# Autodesk Inventor assembly: Linear Actuator
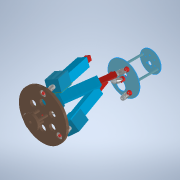
[picture p0: Inventor's stored thumbnail of the model, 180x180]
Saved by Autodesk Inventor 2021 (Build 250183000, 183)
## iProperties
Created: 2021-08-22
Part Number: Linear Actuator
Document SubType Name: Assembly
Designer: techv
Mass: 1736.04 g
Surface Area: 2681.18 cm^2
Volume: 406.885 cm^3
Density: 4.26665 g/cm^3
Author: techv
## Documents named in this file (17)
- D:\Projects\P_Borewell\V3\Linear Actuator.iam
- D:\Projects\P_Borewell\V3\Cylinder.ipt
- D:\Projects\P_Borewell\V3\plunger.ipt
- D:\Projects\P_Borewell\V3\lead screw.ipt
- D:\Projects\P_Borewell\V3\BRACKET N-20 motor v2_Predeterminado.ipt
- D:\Projects\P_Borewell\V3\MicroGearmotor v3.ipt.ipt
- D:\Projects\P_Borewell\V3\as 1420 - 1973 - m3 x 6.ipt
- D:\Projects\P_Borewell\V3\Part5^Assem1 N20 motor and flange.ipt
- D:\Projects\P_Borewell\V2\Design\sps manipulator\coupler.ipt
- D:\Projects\P_Borewell\V2\Design\sps manipulator\Bearing3.iam
- C:\Users\techv\Documents\Inventor\Content Center Files\R2021\en-US\AS 1474(1)\AS 1474 - M6(1).ipt
- C:\Users\techv\Documents\Capsule.ipt
- D:\Projects\P_Borewell\V2\Design\sps manipulator\Craftsman Socket U-Joint_2.iam
- D:\Projects\P_Borewell\V2\Design\sps manipulator\female joint for uv.ipt
- D:\Projects\P_Borewell\V2\Design\sps manipulator\base.ipt
- D:\Projects\P_Borewell\V2\Design\sps manipulator\platform.ipt
- MicroGearmotor v3.ipt
## Components (57 placed, 15 different names)
1. Cylinder:1 — Flush:1, Angle:1, Mate:19, Mate:25, Mate:35, Flush:6, Mate:36, Flush:7, Mate:61, Mate:62
2. plunger:1 — Mate:25, Flush:5, Mate:33, Mate:34, Mate:36, Mate:132, Mate:133
3. lead screw:1 — Flush:1, Mate:16, Mate:31, Mate:33
4. BRACKET N-20 motor v2_Predeterminado:1 — Flush:2, Mate:5, Mate:6, Mate:8, Mate:11, Mate:14, Mate:15
5. MicroGearmotor v3.ipt:1 — Mate:11, Mate:12, Mate:13, Mate:16, Mate:17, Mate:18
6. as 1420 - 1973 - m3 x 6:1 — Mate:5, Mate:6, Mate:7
7. as 1420 - 1973 - m3 x 6:2 — Mate:10, Mate:14, Mate:15
8. Part5^Assem1 N20 motor and flange:1 — Flush:2, Mate:7, Mate:8, Mate:10, Mate:12, Mate:13, Angle:1
9. coupler:1 — Mate:17, Mate:18, Mate:19, Mate:20
10. Bearing3:1 [sub-assembly] — Mate:20, Mate:35, Flush:6
11. AS 1474 - Metric M6:1 — Mate:31, Flush:5, Mate:34
12. Capsule:1 — Flush:7, Mate:60, Mate:61, Mate:62, Mate:109
13. Craftsman Socket U-Joint_2:2 [sub-assembly] — Mate:44, Mate:45, Mate:54, Mate:58
14. female joint for uv:4 — Mate:44, Mate:45, Mate:111, Mate:113
15. base:1 — Mate:37, Mate:38, Mate:39, Flush:8, Flush:9, Flush:10, Mate:55, Mate:57, Mate:58, Mate:59
16. Bearing3:2 [sub-assembly] — Mate:39, Flush:8, Mate:54
17. Bearing3:3 [sub-assembly] — Mate:38, Flush:10, Mate:53
18. Bearing3:4 [sub-assembly] — Mate:37, Flush:9, Mate:52, Mate:56
19. Craftsman Socket U-Joint_2:8 [sub-assembly] — Mate:55, Mate:57
20. female joint for uv:5
21. Craftsman Socket U-Joint_2:9 [sub-assembly] — Mate:52, Mate:56
22. female joint for uv:6 — Mate:60, Mate:109
23. Craftsman Socket U-Joint_2:10 [sub-assembly] — Mate:53, Mate:59
24. female joint for uv:7 — Mate:110, Mate:112
25. Cylinder:2
26. plunger:2 — Mate:130, Mate:131
27. lead screw:2
28. BRACKET N-20 motor v2_Predeterminado:2
29. MicroGearmotor v3.ipt:2
30. as 1420 - 1973 - m3 x 6:3
31. as 1420 - 1973 - m3 x 6:4
32. Part5^Assem1 N20 motor and flange:2
33. coupler:2
34. Bearing3:5 [sub-assembly]
35. AS 1474 - Metric M6:2
36. Capsule:2 — Mate:110, Mate:112
37. Cylinder:3
38. plunger:3 — Mate:134
39. lead screw:3
40. BRACKET N-20 motor v2_Predeterminado:3
41. MicroGearmotor v3.ipt:3
42. as 1420 - 1973 - m3 x 6:5
43. as 1420 - 1973 - m3 x 6:6
44. Part5^Assem1 N20 motor and flange:3
45. coupler:3
46. Bearing3:6 [sub-assembly]
47. AS 1474 - Metric M6:3
48. Capsule:3 — Mate:111, Mate:113
49. platform:1 — Mate:120, Mate:121, Mate:122, Mate:123, Mate:124, Mate:125, Mate:128, Mate:129
50. Craftsman Socket U-Joint_2:11 [sub-assembly] — Mate:122, Mate:123
51. female joint for uv:8 — Mate:132, Mate:133
52. Craftsman Socket U-Joint_2:12 [sub-assembly] — Mate:121, Mate:125
53. female joint for uv:9 — Mate:134
54. Craftsman Socket U-Joint_2:13 [sub-assembly] — Mate:120, Mate:124
55. female joint for uv:10 — Mate:130, Mate:131
56. Craftsman Socket U-Joint_2:14 [sub-assembly] — Mate:128, Mate:129
57. female joint for uv:11
## Relationships (136: Mate 115, Flush 18, Angle 3)
- Flush:1 (-5 mm): Cylinder:1 ↔ lead screw:1
- Flush:2: BRACKET N-20 motor v2_Predeterminado:1 ↔ Part5^Assem1 N20 motor and flange:1
- Mate:5: BRACKET N-20 motor v2_Predeterminado:1 ↔ as 1420 - 1973 - m3 x 6:1
- Mate:6: BRACKET N-20 motor v2_Predeterminado:1 ↔ as 1420 - 1973 - m3 x 6:1
- Mate:7: as 1420 - 1973 - m3 x 6:1 ↔ Part5^Assem1 N20 motor and flange:1
- Mate:8: BRACKET N-20 motor v2_Predeterminado:1 ↔ Part5^Assem1 N20 motor and flange:1
- Mate:10: as 1420 - 1973 - m3 x 6:2 ↔ Part5^Assem1 N20 motor and flange:1
- Mate:11: BRACKET N-20 motor v2_Predeterminado:1 ↔ MicroGearmotor v3.ipt:1
- Mate:12: MicroGearmotor v3.ipt:1 ↔ Part5^Assem1 N20 motor and flange:1
- Mate:13: MicroGearmotor v3.ipt:1 ↔ Part5^Assem1 N20 motor and flange:1
- Mate:14: BRACKET N-20 motor v2_Predeterminado:1 ↔ as 1420 - 1973 - m3 x 6:2
- Mate:15: BRACKET N-20 motor v2_Predeterminado:1 ↔ as 1420 - 1973 - m3 x 6:2
- Mate:16: lead screw:1 ↔ MicroGearmotor v3.ipt:1
- Angle:1 (0 deg): Cylinder:1 ↔ Part5^Assem1 N20 motor and flange:1
- Mate:17 (3 mm): MicroGearmotor v3.ipt:1 ↔ coupler:1
- Mate:18: MicroGearmotor v3.ipt:1 ↔ coupler:1
- Mate:19 (-5 mm): Cylinder:1 ↔ coupler:1
- Mate:20: coupler:1 ↔ Bearing3:1
- Mate:25: Cylinder:1 ↔ plunger:1
- Mate:31: lead screw:1 ↔ AS 1474 - Metric M6:1
- Flush:5: plunger:1 ↔ AS 1474 - Metric M6:1
- Mate:33: plunger:1 ↔ lead screw:1
- Mate:34: plunger:1 ↔ AS 1474 - Metric M6:1
- Mate:35: Cylinder:1 ↔ Bearing3:1
- Flush:6: Cylinder:1 ↔ Bearing3:1
- Mate:36: Cylinder:1 ↔ plunger:1
- Flush:7: Cylinder:1 ↔ Capsule:1
- Mate:37: base:1 ↔ Bearing3:4
- Mate:38: base:1 ↔ Bearing3:3
- Mate:39: base:1 ↔ Bearing3:2
- Flush:8: base:1 ↔ Bearing3:2
- Flush:9: base:1 ↔ Bearing3:4
- Flush:10: base:1 ↔ Bearing3:3
- Mate:44: Craftsman Socket U-Joint_2:2 ↔ female joint for uv:4
- Mate:45: Craftsman Socket U-Joint_2:2 ↔ female joint for uv:4
- [Mate]: Craftsman Socket U-Joint_2:8 ↔ female joint for uv:5
- [Mate]: Craftsman Socket U-Joint_2:8 ↔ female joint for uv:5
- [Mate]: Craftsman Socket U-Joint_2:9 ↔ female joint for uv:6
- [Mate]: Craftsman Socket U-Joint_2:9 ↔ female joint for uv:6
- [Mate]: Craftsman Socket U-Joint_2:10 ↔ female joint for uv:7
- [Mate]: Craftsman Socket U-Joint_2:10 ↔ female joint for uv:7
- Mate:52: Bearing3:4 ↔ Craftsman Socket U-Joint_2:9
- Mate:53: Bearing3:3 ↔ Craftsman Socket U-Joint_2:10
- Mate:54: Craftsman Socket U-Joint_2:2 ↔ Bearing3:2
- Mate:55: base:1 ↔ Craftsman Socket U-Joint_2:8
- Mate:56: Bearing3:4 ↔ Craftsman Socket U-Joint_2:9
- Mate:57: base:1 ↔ Craftsman Socket U-Joint_2:8
- Mate:58: Craftsman Socket U-Joint_2:2 ↔ base:1
- Mate:59: base:1 ↔ Craftsman Socket U-Joint_2:10
- Mate:60: Capsule:1 ↔ female joint for uv:6
- Mate:61: Cylinder:1 ↔ Capsule:1
- Mate:62: Cylinder:1 ↔ Capsule:1
- [Flush] (-5 mm): Cylinder:2 ↔ lead screw:2
- [Flush]: BRACKET N-20 motor v2_Predeterminado:2 ↔ Part5^Assem1 N20 motor and flange:2
- [Mate]: BRACKET N-20 motor v2_Predeterminado:2 ↔ as 1420 - 1973 - m3 x 6:3
- [Mate]: BRACKET N-20 motor v2_Predeterminado:2 ↔ as 1420 - 1973 - m3 x 6:3
- [Mate]: as 1420 - 1973 - m3 x 6:3 ↔ Part5^Assem1 N20 motor and flange:2
- [Mate]: BRACKET N-20 motor v2_Predeterminado:2 ↔ Part5^Assem1 N20 motor and flange:2
- [Mate]: as 1420 - 1973 - m3 x 6:4 ↔ Part5^Assem1 N20 motor and flange:2
- [Mate]: BRACKET N-20 motor v2_Predeterminado:2 ↔ MicroGearmotor v3.ipt:2
- [Mate]: MicroGearmotor v3.ipt:2 ↔ Part5^Assem1 N20 motor and flange:2
- [Mate]: MicroGearmotor v3.ipt:2 ↔ Part5^Assem1 N20 motor and flange:2
- [Mate]: BRACKET N-20 motor v2_Predeterminado:2 ↔ as 1420 - 1973 - m3 x 6:4
- [Mate]: BRACKET N-20 motor v2_Predeterminado:2 ↔ as 1420 - 1973 - m3 x 6:4
- [Mate]: lead screw:2 ↔ MicroGearmotor v3.ipt:2
- [Angle] (0 deg): Cylinder:2 ↔ Part5^Assem1 N20 motor and flange:2
- [Mate] (3 mm): MicroGearmotor v3.ipt:2 ↔ coupler:2
- [Mate]: MicroGearmotor v3.ipt:2 ↔ coupler:2
- [Mate] (-5 mm): Cylinder:2 ↔ coupler:2
- [Mate]: coupler:2 ↔ Bearing3:5
- [Mate]: Cylinder:2 ↔ plunger:2
- [Mate]: lead screw:2 ↔ AS 1474 - Metric M6:2
- [Flush]: plunger:2 ↔ AS 1474 - Metric M6:2
- [Mate]: plunger:2 ↔ lead screw:2
- [Mate]: plunger:2 ↔ AS 1474 - Metric M6:2
- [Mate]: Cylinder:2 ↔ Bearing3:5
- [Flush]: Cylinder:2 ↔ Bearing3:5
- [Mate]: Cylinder:2 ↔ plunger:2
- [Flush]: Cylinder:2 ↔ Capsule:2
- [Mate]: Cylinder:2 ↔ Capsule:2
- [Mate]: Cylinder:2 ↔ Capsule:2
- [Flush] (-5 mm): Cylinder:3 ↔ lead screw:3
- [Flush]: BRACKET N-20 motor v2_Predeterminado:3 ↔ Part5^Assem1 N20 motor and flange:3
- [Mate]: BRACKET N-20 motor v2_Predeterminado:3 ↔ as 1420 - 1973 - m3 x 6:5
- [Mate]: BRACKET N-20 motor v2_Predeterminado:3 ↔ as 1420 - 1973 - m3 x 6:5
- [Mate]: as 1420 - 1973 - m3 x 6:5 ↔ Part5^Assem1 N20 motor and flange:3
- [Mate]: BRACKET N-20 motor v2_Predeterminado:3 ↔ Part5^Assem1 N20 motor and flange:3
- [Mate]: as 1420 - 1973 - m3 x 6:6 ↔ Part5^Assem1 N20 motor and flange:3
- [Mate]: BRACKET N-20 motor v2_Predeterminado:3 ↔ MicroGearmotor v3.ipt:3
- [Mate]: MicroGearmotor v3.ipt:3 ↔ Part5^Assem1 N20 motor and flange:3
- [Mate]: MicroGearmotor v3.ipt:3 ↔ Part5^Assem1 N20 motor and flange:3
- [Mate]: BRACKET N-20 motor v2_Predeterminado:3 ↔ as 1420 - 1973 - m3 x 6:6
- [Mate]: BRACKET N-20 motor v2_Predeterminado:3 ↔ as 1420 - 1973 - m3 x 6:6
- [Mate]: lead screw:3 ↔ MicroGearmotor v3.ipt:3
- [Angle] (0 deg): Cylinder:3 ↔ Part5^Assem1 N20 motor and flange:3
- [Mate] (3 mm): MicroGearmotor v3.ipt:3 ↔ coupler:3
- [Mate]: MicroGearmotor v3.ipt:3 ↔ coupler:3
- [Mate] (-5 mm): Cylinder:3 ↔ coupler:3
- [Mate]: coupler:3 ↔ Bearing3:6
- [Mate]: Cylinder:3 ↔ plunger:3
- [Mate]: lead screw:3 ↔ AS 1474 - Metric M6:3
- [Flush]: plunger:3 ↔ AS 1474 - Metric M6:3
- [Mate]: plunger:3 ↔ lead screw:3
- [Mate]: plunger:3 ↔ AS 1474 - Metric M6:3
- [Mate]: Cylinder:3 ↔ Bearing3:6
- [Flush]: Cylinder:3 ↔ Bearing3:6
- [Mate]: Cylinder:3 ↔ plunger:3
- [Flush]: Cylinder:3 ↔ Capsule:3
- [Mate]: Cylinder:3 ↔ Capsule:3
- [Mate]: Cylinder:3 ↔ Capsule:3
- Mate:109: Capsule:1 ↔ female joint for uv:6
- Mate:110: female joint for uv:7 ↔ Capsule:2
- Mate:111: female joint for uv:4 ↔ Capsule:3
- Mate:112: female joint for uv:7 ↔ Capsule:2
- Mate:113: female joint for uv:4 ↔ Capsule:3
- [Mate]: Craftsman Socket U-Joint_2:11 ↔ female joint for uv:8
- [Mate]: Craftsman Socket U-Joint_2:11 ↔ female joint for uv:8
- [Mate]: Craftsman Socket U-Joint_2:12 ↔ female joint for uv:9
- [Mate]: Craftsman Socket U-Joint_2:12 ↔ female joint for uv:9
- [Mate]: Craftsman Socket U-Joint_2:13 ↔ female joint for uv:10
- [Mate]: Craftsman Socket U-Joint_2:13 ↔ female joint for uv:10
- Mate:120: platform:1 ↔ Craftsman Socket U-Joint_2:13
- Mate:121: platform:1 ↔ Craftsman Socket U-Joint_2:12
- Mate:122: platform:1 ↔ Craftsman Socket U-Joint_2:11
- Mate:123: platform:1 ↔ Craftsman Socket U-Joint_2:11
- Mate:124: platform:1 ↔ Craftsman Socket U-Joint_2:13
- Mate:125: platform:1 ↔ Craftsman Socket U-Joint_2:12
- [Mate]: Craftsman Socket U-Joint_2:14 ↔ female joint for uv:11
- [Mate]: Craftsman Socket U-Joint_2:14 ↔ female joint for uv:11
- Mate:128: platform:1 ↔ Craftsman Socket U-Joint_2:14
- Mate:129: platform:1 ↔ Craftsman Socket U-Joint_2:14
- Mate:130: plunger:2 ↔ female joint for uv:10
- Mate:131: plunger:2 ↔ female joint for uv:10
- Mate:132: plunger:1 ↔ female joint for uv:8
- Mate:133: plunger:1 ↔ female joint for uv:8
- Mate:134: plunger:3 ↔ female joint for uv:9
## Named parameters: d67_d65 = 0 mm, d68_d66 = 0 mm, d69_d65 = 0 mm, d70_d66 = 0 mm, d71_d65 = 0 mm, d72_d66 = 0 mm, d84_d82 = 0 mm, d85_d83 = 0 mm, d86_d3 = -5 mm, d87_d37 = 0 mm, d88_d43 = 0 mm, d89_d45 = 0 mm, d90_d47 = 0 mm, d91_d48 = 0 mm, d92_d49 = 0 mm, d93_d50 = 0 mm, d94_d51 = 0 mm, d95_d54 = 0 mm, d96_d9 = 0 mm, d97_d10 = 0 mm, d98_d11 = 0 mm, d99_d12 = 0 mm, d100_d13 = 0 mm, d101_d15 = 0 mm, d102_d16 = 0 mm, d103_d17 = 0 mm, d104_d18 = 0 mm, d105_d19 = 0 mm, d106_d20 = 0 mm, d107_d21 = 0 mm, d108_d22 = 0 deg, d109_d23 = 3 mm, d110_d24 = 0 mm, d111_d25 = -5 mm, d112_d27 = 0 mm, d113_d35 = 0 mm, d114_d36 = 90 mm, d115_d82 = 0 mm, d116_d83 = 0 mm, d117_d3 = -5 mm, d118_d37 = 0 mm, d119_d43 = 0 mm, d120_d45 = 0 mm, d121_d47 = 0 mm, d122_d48 = 0 mm, d123_d49 = 0 mm, d124_d50 = 0 mm, d125_d51 = 0 mm, d126_d54 = 0 mm, d127_d9 = 0 mm, d128_d10 = 0 mm, d129_d11 = 0 mm, d130_d12 = 0 mm, d131_d13 = 0 mm, d132_d15 = 0 mm, d133_d16 = 0 mm, d134_d17 = 0 mm, d135_d18 = 0 mm, d136_d19 = 0 mm, d137_d20 = 0 mm, d138_d21 = 0 mm, d139_d22 = 0 deg, d140_d23 = 3 mm, d141_d24 = 0 mm, d142_d25 = -5 mm, d143_d27 = 0 mm, d144_d35 = 0 mm, d145_d36 = 90 mm, d182_d67_d65 = 0 mm, d183_d68_d66 = 0 mm, d184_d67_d65 = 0 mm, d185_d68_d66 = 0 mm, d186_d67_d65 = 0 mm, d187_d68_d66 = 0 mm, d194_d67_d65 = 0 mm, d195_d68_d66 = 0 mm
